# Autodesk Inventor assembly: EnsamblajeKNIGHT COMPLETO
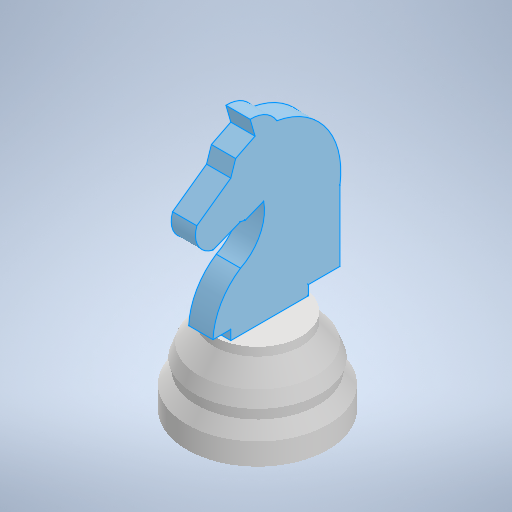
[picture p0: Inventor's stored thumbnail of the model, 512x512]
Saved by Autodesk Inventor 2025.1 (Build 291241000, 241)
## iProperties
Created: 2024-10-24
Part Number: EnsamblajeKNIGHT COMPLETO
Document SubType Name: Assembly
Designer: Octavio
Author: Octavio
## Documents named in this file (3)
- C:\Users\Octavio\Documents\Inventor\CABALLO\ENSAMBLAJE KNIGHT\EnsamblajeKNIGHT COMPLETO.iam
- C:\Users\Octavio\Documents\Inventor\CABALLO\KIGTH TOP 1.0.ipt
- C:\Users\Octavio\Documents\Inventor\CABALLO\KINGHT BASE 1.0.ipt
## Components (2 placed, 2 different names)
1. KIGTH TOP 1.0:1 — Rígido:1
2. KINGHT BASE 1.0:1 — Rígido:1
## Relationships (1: WeldJoint 1)
- Rígido:1 [WeldJoint]: KIGTH TOP 1.0:1 ↔ KINGHT BASE 1.0:1
